# Autodesk Inventor assembly: Gluecksrad_gesamt
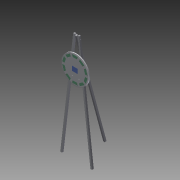
[picture p0: Inventor's stored thumbnail of the model, 180x180]
Saved by Autodesk Inventor 2015 (Build 190159000, 159)
## iProperties
Created: 2018-03-07
Part Number: Gluecksrad_gesamt
Document SubType Name: Assembly
Designer: wepet
Author: Peter Weissig
## Documents named in this file (8)
- C:\workspace\robosax\gluecksrad\Gluecksrad_gesamt.iam
- C:\workspace\robosax\gluecksrad\Grundplatte.ipt
- C:\workspace\robosax\gluecksrad\Platine_led.ipt
- C:\workspace\robosax\gluecksrad\Platine_MCU.ipt
- C:\workspace\robosax\gluecksrad\Plexiglas.ipt
- C:\workspace\robosax\gluecksrad\Standbein_aussen.ipt
- C:\workspace\robosax\gluecksrad\Standbein_mitte.ipt
- C:\workspace\robosax\gluecksrad\Zusatzelemente\licht_taster.ipt
## Components (18 placed, 7 different names)
1. Grundplatte:1 — Passend:1, Passend:2, Passend:3, Passend:4, Passend:5, Passend:6, Passend:7, Passend:8, Passend:9, Passend:10, Passend:12, Passend:13, Passend:14, Passend:17, Winkel:1
2. Platine_MCU:1 — Passend:2, Passend:3, Passend:4, Passend:11, Fluchtend:2
3. Plexiglas:1 — Passend:8, Passend:9, Passend:10
4. Standbein_aussen:1 — Passend:14, Passend:16, Passend:19, Passend:20
5. Standbein_mitte:1 — Passend:16, Passend:18, Winkel:1, Fluchtend:1, Passend:20
6. licht_taster:1 — Passend:13
7. licht_taster:2 — Passend:12
8. Standbein_aussen:2 — Passend:17, Passend:18, Passend:19, Passend:21
9. Platine_led:1 — Passend:5, Passend:6, Passend:7
10. Platine_led:2
11. Platine_led:3
12. Platine_led:4
13. Platine_led:5
14. Platine_led:6
15. Platine_led:7
16. Platine_led:8
17. Platine_led:9
18. Platine_led:10
## Component patterns: (10 elements, first: Platine_led:1)
## Relationships (23: Mate 20, Flush 2, Angle 1)
- Passend:1 [Mate]: Grundplatte:1
- Passend:2 [Mate] (10 mm): Grundplatte:1 ↔ Platine_MCU:1
- Passend:3 [Mate] (10 mm): Grundplatte:1 ↔ Platine_MCU:1
- Passend:4 [Mate] (10 mm): Grundplatte:1 ↔ Platine_MCU:1
- Passend:5 [Mate] (10 mm): Grundplatte:1 ↔ Platine_led:1
- Passend:6 [Mate] (10 mm): Grundplatte:1 ↔ Platine_led:1
- Passend:7 [Mate] (10 mm): Grundplatte:1 ↔ Platine_led:1
- Passend:8 [Mate] (18 mm): Grundplatte:1 ↔ Plexiglas:1
- Passend:9 [Mate]: Grundplatte:1 ↔ Plexiglas:1
- Passend:10 [Mate]: Grundplatte:1 ↔ Plexiglas:1
- Passend:11 [Mate] (-40 mm): Platine_MCU:1
- Passend:12 [Mate]: Grundplatte:1 ↔ licht_taster:2
- Passend:13 [Mate]: Grundplatte:1 ↔ licht_taster:1
- Passend:14 [Mate]: Grundplatte:1 ↔ Standbein_aussen:1
- Passend:16 [Mate]: Standbein_aussen:1 ↔ Standbein_mitte:1
- Passend:17 [Mate]: Grundplatte:1 ↔ Standbein_aussen:2
- Passend:18 [Mate]: Standbein_mitte:1 ↔ Standbein_aussen:2
- Winkel:1 [Angle] (15 deg): Grundplatte:1 ↔ Standbein_mitte:1
- Fluchtend:1 [Flush] (-15 mm): Standbein_mitte:1
- Fluchtend:2 [Flush] (-50 mm): Platine_MCU:1
- Passend:19 [Mate] (50 mm): Standbein_aussen:1 ↔ Standbein_aussen:2
- Passend:20 [Mate] (19 mm): Standbein_aussen:1 ↔ Standbein_mitte:1
- Passend:21 [Mate] (-1450 mm): Standbein_aussen:2
